# Autodesk Inventor assembly: ensambleOrigen
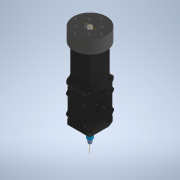
[picture p0: Inventor's stored thumbnail of the model, 180x180]
Saved by Autodesk Inventor 2021.5 (Build 255421000, 421)
## iProperties
Created: 2024-11-29
Part Number: ensambleOrigen
Document SubType Name: Assembly
Designer: Joho_
Mass: 149.614 g
Surface Area: 563.762 cm^2
Volume: 135.167 cm^3
Density: 1.10688 g/cm^3
Author: Joho_
## Documents named in this file (2)
- C:\Users\Joho_\Desktop\semestreN\robotica\laboratorios\lab01\CADs\ensambleOrigen.iam
- C:\Users\Joho_\Desktop\semestreN\robotica\laboratorios\lab01\CADs\ensambleSinFlanche.iam
## Components (1 placed, 1 different names)
1. ensambleSinFlanche:1 [sub-assembly] — Coincidencia:1, Coincidencia:2, Coincidencia:3, Nivelación:1
## Relationships (4: Mate 3, Flush 1)
- Coincidencia:1 [Mate]: ensambleSinFlanche:1
- Coincidencia:2 [Mate]: ensambleSinFlanche:1
- Coincidencia:3 [Mate]: ensambleSinFlanche:1
- Nivelación:1 [Flush]: ensambleSinFlanche:1
